# Autodesk Inventor assembly: Prototipo 2
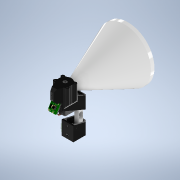
[picture p0: Inventor's stored thumbnail of the model, 180x180]
Saved by Autodesk Inventor 2022 (Build 260153000, 153)
## iProperties
Created: 2021-02-18
Part Number: Prototipo 2
Document SubType Name: Assembly
Designer: juanp
Author: juanp
## Documents named in this file (12)
- C:\Users\juanp\Desktop\Robocol\EVA\V3 (Actual)\Dispensador\Dispensador V2.iam
- C:\Users\juanp\Desktop\Robocol\EVA\Recursos\Servo MG996R\Servo Motor MG996R.iam
- C:\Users\juanp\Desktop\Robocol\EVA\V3 (Actual)\Dispensador\attachmentcustom.ipt
- C:\Users\juanp\Desktop\Robocol\EVA\V3 (Actual)\Dispensador\Valvula.ipt
- C:\Users\juanp\Desktop\Robocol\EVA\V3 (Actual)\Dispensador\Retenedor.ipt
- C:\Users\juanp\Desktop\Robocol\EVA\V3 (Actual)\Dispensador\Carcasa.ipt
- C:\Users\juanp\Desktop\Robocol\EVA\Recursos\Celda de Carga\CELDA DE PRESION ARDUINO.ipt
- C:\Users\juanp\Desktop\Robocol\EVA\V3 (Actual)\Dispensador\Soporte Actuador V2.ipt
- C:\Users\juanp\Desktop\Robocol\EVA\V3 (Actual)\Camara\Case.ipt
- C:\Users\juanp\Desktop\Robocol\EVA\Recursos\Pi Camera\RspCameraMia.iam
- C:\Users\juanp\Desktop\Robocol\EVA\V3 (Actual)\Dispensador\Arandela HX711.ipt
- C:\Users\juanp\Desktop\Robocol\EVA\Recursos\HX711\Hx711 Full.ipt
## Components (15 placed, 11 different names)
1. Servo Motor MG996R:1 [sub-assembly] — Mate:1, Mate:2, Flush:1, Mate:3, Mate:4, Mate:11
2. attachmentcustom:1 — Mate:3, Mate:4, Mate:5, Mate:6, Flush:2, Flush:3, Mate:21, Mate:22
3. Valvula:1 — Mate:5, Mate:7, Mate:8, Mate:21
4. Retenedor:1 — Mate:6, Mate:7, Flush:2
5. Retenedor:2 — Mate:8
6. Carcasa:1 — Flush:3, Mate:11, Mate:22, Mate:23, Mate:24, Mate:25, Mate:29, Flush:4, Flush:5
7. CELDA DE PRESION ARDUINO:1 — Mate:23, Mate:24, Mate:25, Mate:26, Mate:27, Mate:28
8. Soporte Actuador V2:1 — Mate:26, Mate:27, Mate:28, Mate:33, Mate:34, Mate:35
9. Case:1 — Mate:29, Mate:30, Mate:31, Mate:32, Flush:5
10. RspCameraMia:1 [sub-assembly] — Mate:30, Mate:31, Mate:32, Flush:4
11. Arandela HX711:1 — Flush:6, Mate:34, Mate:36, Mate:39
12. Arandela HX711:2 — Flush:6, Mate:33, Mate:35, Mate:37, Mate:38
13. Arandela HX711:3 — Flush:7, Mate:39
14. Arandela HX711:4 — Flush:7, Mate:40, Mate:41
15. Hx711 Full:1 — Mate:36, Mate:37, Mate:38, Mate:40, Mate:41
## Relationships (37: Mate 30, Flush 7)
- Mate:1: Servo Motor MG996R:1
- Mate:2: Servo Motor MG996R:1
- Flush:1: Servo Motor MG996R:1
- Mate:3: Servo Motor MG996R:1 ↔ attachmentcustom:1
- Mate:4: Servo Motor MG996R:1 ↔ attachmentcustom:1
- Mate:5: attachmentcustom:1 ↔ Valvula:1
- Mate:6: attachmentcustom:1 ↔ Retenedor:1
- Mate:7: Valvula:1 ↔ Retenedor:1
- Mate:8: Valvula:1 ↔ Retenedor:2
- Flush:2 (2.5 mm): attachmentcustom:1 ↔ Retenedor:1
- Flush:3: attachmentcustom:1 ↔ Carcasa:1
- Mate:11: Servo Motor MG996R:1 ↔ Carcasa:1
- Mate:21: attachmentcustom:1 ↔ Valvula:1
- Mate:22: attachmentcustom:1 ↔ Carcasa:1
- Mate:23: Carcasa:1 ↔ CELDA DE PRESION ARDUINO:1
- Mate:24: Carcasa:1 ↔ CELDA DE PRESION ARDUINO:1
- Mate:25: Carcasa:1 ↔ CELDA DE PRESION ARDUINO:1
- Mate:26: CELDA DE PRESION ARDUINO:1 ↔ Soporte Actuador V2:1
- Mate:27: CELDA DE PRESION ARDUINO:1 ↔ Soporte Actuador V2:1
- Mate:28: CELDA DE PRESION ARDUINO:1 ↔ Soporte Actuador V2:1
- Mate:29: Carcasa:1 ↔ Case:1
- Mate:30: Case:1 ↔ RspCameraMia:1
- Mate:31: Case:1 ↔ RspCameraMia:1
- Mate:32: Case:1 ↔ RspCameraMia:1
- Flush:4: Carcasa:1 ↔ RspCameraMia:1
- Flush:5: Carcasa:1 ↔ Case:1
- Flush:6: Arandela HX711:1 ↔ Arandela HX711:2
- Mate:33: Soporte Actuador V2:1 ↔ Arandela HX711:2
- Mate:34: Soporte Actuador V2:1 ↔ Arandela HX711:1
- Mate:35: Soporte Actuador V2:1 ↔ Arandela HX711:2
- Mate:36: Arandela HX711:1 ↔ Hx711 Full:1
- Mate:37: Arandela HX711:2 ↔ Hx711 Full:1
- Mate:38: Arandela HX711:2 ↔ Hx711 Full:1
- Flush:7: Arandela HX711:3 ↔ Arandela HX711:4
- Mate:39: Arandela HX711:1 ↔ Arandela HX711:3
- Mate:40: Arandela HX711:4 ↔ Hx711 Full:1
- Mate:41: Arandela HX711:4 ↔ Hx711 Full:1
